# Autodesk Inventor assembly: WheelAssembly3.0
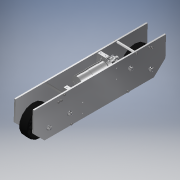
[picture p0: Inventor's stored thumbnail of the model, 180x180]
Saved by Autodesk Inventor 2017 (Build 210142000, 142)
## iProperties
Created: 2017-07-22
Part Number: WheelAssembly3.0
Document SubType Name: Assembly
Designer: User
Mass: 2283.58 g
Surface Area: 3964.96 cm^2
Volume: 891.781 cm^3
Density: 2.56069 g/cm^3
Author: User
## Documents named in this file (19)
- C:\Robotics\CAD\2018-19_CAD\InvertedDriveTrain.iam
- C:\Robotics\CAD\COTSParts\Motors\Andymark 2964  NeveRest 40 Motor.ipt
- C:\Robotics\CAD\COTSParts\Tetrix\tetrix-motor-mounts-1.snapshot.1\Tetrex 2pc motor mount.ipt
- C:\Robotics\CAD\COTSParts\Actobotics\615 parts\615398.25inBoreBeveledGears.ipt
- C:\Robotics\CAD\2016-17_CAD\Custom COTS\4inax.ipt
- C:\Robotics\CAD\COTSParts\Actobotics\615 parts\615106Sprocket.5inBore.25inPitch24Teeth.ipt
- C:\Robotics\CAD\COTSParts\Actobotics\545 parts\545556SetScrewHub.77inPattern.ipt
- C:\Robotics\CAD\COTSParts\Wheels\4in Wheel Intergreated Hub 8mm Rev2.ipt
- C:\Robotics\CAD\COTSParts\Actobotics\Thrust Bearings\6655K13.ipt
- C:\Robotics\CAD\2018-19_CAD\InvertedDrivePlateOutside.ipt
- C:\Robotics\CAD\2018-19_CAD\InvertedDrivePlateInside.ipt
- C:\Robotics\CAD\2018-19_CAD\Offseason\WheelandSprocketComboHub2.ipt
- C:\Robotics\CAD\COTSParts\Actobotics\535 parts\535198Bearing.25ID.5OD.ipt
- C:\Robotics\CAD\2018-19_CAD\Offseason\Tensioner3.iam
- C:\Robotics\CAD\2018-19_CAD\Offseason\MotorFixedPositionMountInvertedDrive.ipt
- C:\Robotics\CAD\COTSParts\Actobotics\Collar.ipt
- C:\Robotics\CAD\COTSParts\Fasteners\6-32 SHCS x500.ipt
- C:\Robotics\CAD\COTSParts\Fasteners\6-32 SHCS x250.ipt
- C:\Robotics\CAD\COTSParts\Fasteners\Hex Standoff 6-32 x2250.ipt
## Components (84 placed, 18 different names)
1. Andymark 2964  NeveRest 40 Motor:1 — Insert:3, Insert:6, Angle:13
2. Andymark 2964  NeveRest 40 Motor:2 — Insert:4, Insert:5, Angle:14
3. Tetrex 2pc motor mount:1 — Insert:3, Insert:79, Angle:8, Insert:84, Angle:13
4. Tetrex 2pc motor mount:2 — Insert:4, Insert:80, Angle:9, Insert:85, Angle:14
5. 615398.25inBoreBeveledGears:1 — Insert:5, Insert:44, Rotation:5
6. 615398.25inBoreBeveledGears:2 — Insert:6, Insert:47, Rotation:8
7. 615398.25inBoreBeveledGears:3 — Insert:77, Rotation:7, Rotation:8
8. 615398.25inBoreBeveledGears:4 — Insert:78, Rotation:4, Rotation:5
9. 4inax:1 — Mate:34, Insert:146
10. 4inax:2 — Insert:145
11. 615106Sprocket.5inBore.25inPitch24Teeth:2 — Insert:102, Insert:103, Insert:104, Flush:3, Rotation:6
12. 4inax:3 — Mate:33, Insert:144
13. 4inax:4 — Insert:147
14. 545556SetScrewHub.77inPattern:4 — Insert:110, Insert:111, Mate:33
15. 4in Wheel Intergreated Hub 8mm Rev2:1 — Insert:65, Insert:126, Insert:127, Rotation:2
16. 4in Wheel Intergreated Hub 8mm Rev2:2 — Insert:68, Insert:124, Insert:125, Rotation:1
17. 545556SetScrewHub.77inPattern:7 — Insert:114, Insert:115
18. 615106Sprocket.5inBore.25inPitch24Teeth:3 — Insert:105, Insert:106, Insert:107, Flush:4, Rotation:3
19. 6655K13:1 — Insert:64, Insert:78
20. 6655K13:2 — Insert:63, Insert:77
21. 6655K13:3 — Insert:44
22. 6655K13:4 — Insert:47
23. 615106Sprocket.5inBore.25inPitch24Teeth:4 — Insert:108, Insert:109, Insert:110, Insert:111, Flush:3, Rotation:6, Rotation:7
24. 615106Sprocket.5inBore.25inPitch24Teeth:5 — Insert:112, Insert:113, Insert:114, Insert:115, Mate:34, Flush:4, Rotation:3, Rotation:4
25. InvertedDrivePlateOutside:1 — Insert:71, Insert:72, Insert:73, Insert:74, Insert:75, Insert:76, Angle:10, Insert:81, Insert:82, Insert:83, Insert:116, Insert:117, Insert:118, Insert:119, Insert:128, Insert:129, Insert:130, Insert:131, Insert:136, Insert:137, Insert:138, Insert:139
26. InvertedDrivePlateInside:1 — Insert:63, Insert:64, Insert:79, Angle:8, Insert:80, Angle:9, Angle:11, Angle:12, Insert:90, Insert:91, Insert:92, Insert:93, Insert:98, Insert:99, Insert:100, Insert:101, Insert:132, Insert:133, Insert:134, Insert:135, Insert:140, Insert:141, Insert:142, Insert:143
27. WheelandSprocketComboHub2:1 — Insert:68, Insert:75, Insert:104, Mate:31, Rotation:1
28. WheelandSprocketComboHub2:2 — Insert:65, Insert:76, Insert:107, Mate:32, Rotation:2
29. 535198Bearing.25ID.5OD:1 — Insert:71, Insert:86
30. 535198Bearing.25ID.5OD:2 — Insert:74, Insert:89
31. 535198Bearing.25ID.5OD:3 — Insert:73, Insert:88
32. 535198Bearing.25ID.5OD:4 — Insert:72, Insert:87
33. Tensioner3:1 [sub-assembly] — Insert:82, Insert:83
34. Tensioner3:2 [sub-assembly] — Angle:10, Insert:81
35. MotorFixedPositionMountInvertedDrive:1 — Insert:84, Angle:11, Insert:120, Insert:121
36. MotorFixedPositionMountInvertedDrive:2 — Insert:85, Angle:12, Insert:122, Insert:123
37. Collar:1 — Insert:86, Insert:147
38. Collar:2 — Insert:87, Insert:144
39. Collar:3 — Insert:88, Insert:146
40. Collar:4 — Insert:89, Insert:145
41. Collar:5 — Insert:97
42. Collar:6 — Insert:96
43. Collar:7 — Insert:95
44. Collar:8 — Insert:94
45. 535198Bearing.25ID.5OD:5 — Insert:90, Insert:94
46. 535198Bearing.25ID.5OD:6 — Insert:91, Insert:95
47. 535198Bearing.25ID.5OD:7 — Insert:92, Insert:96
48. 535198Bearing.25ID.5OD:8 — Insert:93, Insert:97
49. 6-32 SHCS x500:1 — Insert:99
50. 6-32 SHCS x500:2 — Insert:98
51. 6-32 SHCS x500:3 — Insert:100
52. 6-32 SHCS x500:4 — Insert:101
53. 6-32 SHCS x500:5 — Insert:105, Mate:32
54. 6-32 SHCS x500:6 — Insert:106
55. 6-32 SHCS x500:7 — Insert:103
56. 6-32 SHCS x500:9 — Insert:102, Mate:31
57. 6-32 SHCS x250:1 — Insert:108
58. 6-32 SHCS x250:2 — Insert:109
59. 6-32 SHCS x250:3 — Insert:113
60. 6-32 SHCS x250:4 — Insert:112
61. 6-32 SHCS x500:10 — Insert:117
62. 6-32 SHCS x500:11 — Insert:116
63. 6-32 SHCS x500:12 — Insert:118
64. 6-32 SHCS x500:13 — Insert:119
65. 6-32 SHCS x500:14 — Insert:120
66. 6-32 SHCS x500:15 — Insert:121
67. 6-32 SHCS x500:16 — Insert:123
68. 6-32 SHCS x500:17 — Insert:122
69. 6-32 SHCS x500:18 — Insert:125
70. 6-32 SHCS x500:19 — Insert:124
71. 6-32 SHCS x500:20 — Insert:127
72. 6-32 SHCS x500:21 — Insert:126
73. Hex Standoff 6-32 x2250:1 — Insert:129, Insert:134
74. Hex Standoff 6-32 x2250:2 — Insert:128, Insert:132
75. Hex Standoff 6-32 x2250:3 — Insert:131, Insert:135
76. Hex Standoff 6-32 x2250:4 — Insert:130, Insert:133
77. 6-32 SHCS x500:22 — Insert:136
78. 6-32 SHCS x500:23 — Insert:137
79. 6-32 SHCS x500:24 — Insert:138
80. 6-32 SHCS x500:25 — Insert:139
81. 6-32 SHCS x500:26 — Insert:140
82. 6-32 SHCS x500:27 — Insert:141
83. 6-32 SHCS x500:28 — Insert:142
84. 6-32 SHCS x500:29 — Insert:143
## Relationships (108: Insert 87, RelateRotation 8, Angle 7, Mate 4, Flush 2)
- Insert:3: Andymark 2964  NeveRest 40 Motor:1 ↔ Tetrex 2pc motor mount:1
- Insert:4: Andymark 2964  NeveRest 40 Motor:2 ↔ Tetrex 2pc motor mount:2
- Insert:5: Andymark 2964  NeveRest 40 Motor:2 ↔ 615398.25inBoreBeveledGears:1
- Insert:6: Andymark 2964  NeveRest 40 Motor:1 ↔ 615398.25inBoreBeveledGears:2
- Insert:44: 615398.25inBoreBeveledGears:1 ↔ 6655K13:3
- Insert:47: 615398.25inBoreBeveledGears:2 ↔ 6655K13:4
- Insert:63 (1.4224 mm): 6655K13:2 ↔ InvertedDrivePlateInside:1
- Insert:64 (-1.4224 mm): 6655K13:1 ↔ InvertedDrivePlateInside:1
- Insert:65: 4in Wheel Intergreated Hub 8mm Rev2:1 ↔ WheelandSprocketComboHub2:2
- Insert:68: 4in Wheel Intergreated Hub 8mm Rev2:2 ↔ WheelandSprocketComboHub2:1
- Insert:71: InvertedDrivePlateOutside:1 ↔ 535198Bearing.25ID.5OD:1
- Insert:72: InvertedDrivePlateOutside:1 ↔ 535198Bearing.25ID.5OD:4
- Insert:73: InvertedDrivePlateOutside:1 ↔ 535198Bearing.25ID.5OD:3
- Insert:74: InvertedDrivePlateOutside:1 ↔ 535198Bearing.25ID.5OD:2
- Insert:75 (1.27 mm): InvertedDrivePlateOutside:1 ↔ WheelandSprocketComboHub2:1
- Insert:76 (1.27 mm): InvertedDrivePlateOutside:1 ↔ WheelandSprocketComboHub2:2
- Insert:77: 615398.25inBoreBeveledGears:3 ↔ 6655K13:2
- Insert:78: 615398.25inBoreBeveledGears:4 ↔ 6655K13:1
- Insert:79: Tetrex 2pc motor mount:1 ↔ InvertedDrivePlateInside:1
- Angle:8 (0 deg): Tetrex 2pc motor mount:1 ↔ InvertedDrivePlateInside:1
- Insert:80: Tetrex 2pc motor mount:2 ↔ InvertedDrivePlateInside:1
- Angle:9 (0 deg): Tetrex 2pc motor mount:2 ↔ InvertedDrivePlateInside:1
- Angle:10 (-62 deg): InvertedDrivePlateOutside:1 ↔ Tensioner3:2
- Insert:81: InvertedDrivePlateOutside:1 ↔ Tensioner3:2
- Insert:82: InvertedDrivePlateOutside:1 ↔ Tensioner3:1
- Insert:83: InvertedDrivePlateOutside:1 ↔ Tensioner3:1
- Insert:84: Tetrex 2pc motor mount:1 ↔ MotorFixedPositionMountInvertedDrive:1
- Angle:11 (180 deg): InvertedDrivePlateInside:1 ↔ MotorFixedPositionMountInvertedDrive:1
- Insert:85: Tetrex 2pc motor mount:2 ↔ MotorFixedPositionMountInvertedDrive:2
- Angle:12 (180 deg): InvertedDrivePlateInside:1 ↔ MotorFixedPositionMountInvertedDrive:2
- Insert:86: 535198Bearing.25ID.5OD:1 ↔ Collar:1
- Insert:87: 535198Bearing.25ID.5OD:4 ↔ Collar:2
- Insert:88: 535198Bearing.25ID.5OD:3 ↔ Collar:3
- Insert:89: 535198Bearing.25ID.5OD:2 ↔ Collar:4
- Insert:90: InvertedDrivePlateInside:1 ↔ 535198Bearing.25ID.5OD:5
- Insert:91: InvertedDrivePlateInside:1 ↔ 535198Bearing.25ID.5OD:6
- Insert:92: InvertedDrivePlateInside:1 ↔ 535198Bearing.25ID.5OD:7
- Insert:93: InvertedDrivePlateInside:1 ↔ 535198Bearing.25ID.5OD:8
- Insert:94: Collar:8 ↔ 535198Bearing.25ID.5OD:5
- Insert:95: Collar:7 ↔ 535198Bearing.25ID.5OD:6
- Insert:96: Collar:6 ↔ 535198Bearing.25ID.5OD:7
- Insert:97: Collar:5 ↔ 535198Bearing.25ID.5OD:8
- Insert:98: InvertedDrivePlateInside:1 ↔ 6-32 SHCS x500:2
- Insert:99: InvertedDrivePlateInside:1 ↔ 6-32 SHCS x500:1
- Insert:100: InvertedDrivePlateInside:1 ↔ 6-32 SHCS x500:3
- Insert:101: InvertedDrivePlateInside:1 ↔ 6-32 SHCS x500:4
- Insert:102: 615106Sprocket.5inBore.25inPitch24Teeth:2 ↔ 6-32 SHCS x500:9
- Insert:103: 615106Sprocket.5inBore.25inPitch24Teeth:2 ↔ 6-32 SHCS x500:7
- Insert:104: 615106Sprocket.5inBore.25inPitch24Teeth:2 ↔ WheelandSprocketComboHub2:1
- Mate:31: WheelandSprocketComboHub2:1 ↔ 6-32 SHCS x500:9
- Insert:105: 615106Sprocket.5inBore.25inPitch24Teeth:3 ↔ 6-32 SHCS x500:5
- Insert:106: 615106Sprocket.5inBore.25inPitch24Teeth:3 ↔ 6-32 SHCS x500:6
- Insert:107: 615106Sprocket.5inBore.25inPitch24Teeth:3 ↔ WheelandSprocketComboHub2:2
- Mate:32: WheelandSprocketComboHub2:2 ↔ 6-32 SHCS x500:5
- Insert:108: 615106Sprocket.5inBore.25inPitch24Teeth:4 ↔ 6-32 SHCS x250:1
- Insert:109: 615106Sprocket.5inBore.25inPitch24Teeth:4 ↔ 6-32 SHCS x250:2
- Insert:110: 545556SetScrewHub.77inPattern:4 ↔ 615106Sprocket.5inBore.25inPitch24Teeth:4
- Insert:111: 545556SetScrewHub.77inPattern:4 ↔ 615106Sprocket.5inBore.25inPitch24Teeth:4
- Mate:33: 4inax:3 ↔ 545556SetScrewHub.77inPattern:4
- Flush:3: 615106Sprocket.5inBore.25inPitch24Teeth:2 ↔ 615106Sprocket.5inBore.25inPitch24Teeth:4
- Insert:112: 615106Sprocket.5inBore.25inPitch24Teeth:5 ↔ 6-32 SHCS x250:4
- Insert:113: 615106Sprocket.5inBore.25inPitch24Teeth:5 ↔ 6-32 SHCS x250:3
- Insert:114: 545556SetScrewHub.77inPattern:7 ↔ 615106Sprocket.5inBore.25inPitch24Teeth:5
- Insert:115: 545556SetScrewHub.77inPattern:7 ↔ 615106Sprocket.5inBore.25inPitch24Teeth:5
- Mate:34: 4inax:1 ↔ 615106Sprocket.5inBore.25inPitch24Teeth:5
- Flush:4: 615106Sprocket.5inBore.25inPitch24Teeth:3 ↔ 615106Sprocket.5inBore.25inPitch24Teeth:5
- Insert:116: InvertedDrivePlateOutside:1 ↔ 6-32 SHCS x500:11
- Insert:117: InvertedDrivePlateOutside:1 ↔ 6-32 SHCS x500:10
- Insert:118: InvertedDrivePlateOutside:1 ↔ 6-32 SHCS x500:12
- Insert:119: InvertedDrivePlateOutside:1 ↔ 6-32 SHCS x500:13
- Insert:120: MotorFixedPositionMountInvertedDrive:1 ↔ 6-32 SHCS x500:14
- Insert:121: MotorFixedPositionMountInvertedDrive:1 ↔ 6-32 SHCS x500:15
- Insert:122: MotorFixedPositionMountInvertedDrive:2 ↔ 6-32 SHCS x500:17
- Insert:123: MotorFixedPositionMountInvertedDrive:2 ↔ 6-32 SHCS x500:16
- Angle:13 (0 deg): Andymark 2964  NeveRest 40 Motor:1 ↔ Tetrex 2pc motor mount:1
- Angle:14 (180 deg): Andymark 2964  NeveRest 40 Motor:2 ↔ Tetrex 2pc motor mount:2
- Insert:124: 4in Wheel Intergreated Hub 8mm Rev2:2 ↔ 6-32 SHCS x500:19
- Insert:125: 4in Wheel Intergreated Hub 8mm Rev2:2 ↔ 6-32 SHCS x500:18
- Insert:126: 4in Wheel Intergreated Hub 8mm Rev2:1 ↔ 6-32 SHCS x500:21
- Insert:127: 4in Wheel Intergreated Hub 8mm Rev2:1 ↔ 6-32 SHCS x500:20
- Rotation:1 [RelateRotation] (1 ul): 4in Wheel Intergreated Hub 8mm Rev2:2 ↔ WheelandSprocketComboHub2:1
- Rotation:2 [RelateRotation] (1 ul): 4in Wheel Intergreated Hub 8mm Rev2:1 ↔ WheelandSprocketComboHub2:2
- Rotation:3 [RelateRotation] (1 ul): 615106Sprocket.5inBore.25inPitch24Teeth:3 ↔ 615106Sprocket.5inBore.25inPitch24Teeth:5
- Rotation:4 [RelateRotation] (1 ul): 615398.25inBoreBeveledGears:4 ↔ 615106Sprocket.5inBore.25inPitch24Teeth:5
- Rotation:5 [RelateRotation] (1 ul): 615398.25inBoreBeveledGears:1 ↔ 615398.25inBoreBeveledGears:4
- Rotation:6 [RelateRotation] (1 ul): 615106Sprocket.5inBore.25inPitch24Teeth:2 ↔ 615106Sprocket.5inBore.25inPitch24Teeth:4
- Rotation:7 [RelateRotation] (1 ul): 615398.25inBoreBeveledGears:3 ↔ 615106Sprocket.5inBore.25inPitch24Teeth:4
- Rotation:8 [RelateRotation] (1 ul): 615398.25inBoreBeveledGears:2 ↔ 615398.25inBoreBeveledGears:3
- Insert:128: InvertedDrivePlateOutside:1 ↔ Hex Standoff 6-32 x2250:2
- Insert:129: InvertedDrivePlateOutside:1 ↔ Hex Standoff 6-32 x2250:1
- Insert:130: InvertedDrivePlateOutside:1 ↔ Hex Standoff 6-32 x2250:4
- Insert:131: InvertedDrivePlateOutside:1 ↔ Hex Standoff 6-32 x2250:3
- Insert:132: InvertedDrivePlateInside:1 ↔ Hex Standoff 6-32 x2250:2
- Insert:133: InvertedDrivePlateInside:1 ↔ Hex Standoff 6-32 x2250:4
- Insert:134: InvertedDrivePlateInside:1 ↔ Hex Standoff 6-32 x2250:1
- Insert:135: InvertedDrivePlateInside:1 ↔ Hex Standoff 6-32 x2250:3
- Insert:136: InvertedDrivePlateOutside:1 ↔ 6-32 SHCS x500:22
- Insert:137: InvertedDrivePlateOutside:1 ↔ 6-32 SHCS x500:23
- Insert:138: InvertedDrivePlateOutside:1 ↔ 6-32 SHCS x500:24
- Insert:139: InvertedDrivePlateOutside:1 ↔ 6-32 SHCS x500:25
- Insert:140: InvertedDrivePlateInside:1 ↔ 6-32 SHCS x500:26
- Insert:141: InvertedDrivePlateInside:1 ↔ 6-32 SHCS x500:27
- Insert:142: InvertedDrivePlateInside:1 ↔ 6-32 SHCS x500:28
- Insert:143: InvertedDrivePlateInside:1 ↔ 6-32 SHCS x500:29
- Insert:144: 4inax:3 ↔ Collar:2
- Insert:145: 4inax:2 ↔ Collar:4
- Insert:146: 4inax:1 ↔ Collar:3
- Insert:147: 4inax:4 ↔ Collar:1
